# Autodesk Inventor assembly: カム用ボルトアセンブリ
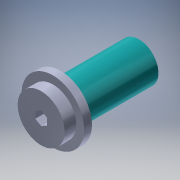
[picture p0: Inventor's stored thumbnail of the model, 180x180]
Saved by Autodesk Inventor 2018 (Build 220112000, 112)
## iProperties
Created: 2018-12-25
Part Number: カム用ボルトアセンブリ
Material: 一般
Document SubType Name: Assembly
Designer: lowyu
Author: lowyu
## Documents named in this file (4)
- C:\Users\lowyu\Desktop\HAND\シャッターハンド\卒論\カム用ボルトアセンブリ.iam
- C:\Users\lowyu\Desktop\HAND\シャッターハンド\内側　支柱.ipt
- C:\Users\lowyu\Desktop\HAND\シャッターハンド\座金.ipt
- C:\Users\lowyu\Desktop\HAND\シャッターハンド\CBSA3-5 極低頭六角穴付ボルト.ipt
## Components (3 placed, 3 different names)
1. 内側　支柱:1 — メイト:1, メイト:4
2. 座金:1 — メイト:2, メイト:3, メイト:4
3. CBSA3-5 極低頭六角穴付ボルト:1 — メイト:1, メイト:2, メイト:3
## Relationships (4: Mate 4)
- メイト:1 [Mate]: 内側　支柱:1 ↔ CBSA3-5 極低頭六角穴付ボルト:1
- メイト:2 [Mate]: 座金:1 ↔ CBSA3-5 極低頭六角穴付ボルト:1
- メイト:3 [Mate]: 座金:1 ↔ CBSA3-5 極低頭六角穴付ボルト:1
- メイト:4 [Mate]: 内側　支柱:1 ↔ 座金:1
